# Autodesk Inventor assembly: m3X20
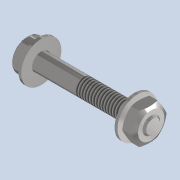
[picture p0: Inventor's stored thumbnail of the model, 180x180]
Saved by Autodesk Inventor 2020 (Build 240168000, 168)
## iProperties
Created: 2021-02-25
Part Number: m3X20
Document SubType Name: Assembly
Designer: Iulian Bors
Author: Iulian Bors
## Documents named in this file (4)
- Z:\I.A.B\Proiecte\0008 I.A.B 3D 2.1 Imprimanta aracet Metal\10 Mecanic\m3X20.iam
- Z:\I.A.B\Proiecte\0008 I.A.B 3D 2.1 Imprimanta aracet Metal\10 Mecanic\0008-10-2004 DIN 7984 - M3 x 20.ipt
- C:\Users\40743\Documents\Inventor\Content Center Files\R2020\en-US\DIN 555\DIN 555-5 - M3.ipt
- Z:\I.A.B\Proiecte\0008 I.A.B 3D 2.1 Imprimanta aracet Metal\10 Mecanic\0008-10-2005 DIN 125 - A 3.2.ipt
## Components (4 placed, 3 different names)
1. 0008-10-2004 DIN 7984 - M3 x 20.ipt:1 — Insert:1, Insert:2
2. DIN 555-5 - M3.ipt:2 — Insert:1, Insert:3
3. 0008-10-2005 DIN 125 - A 3.2.ipt:3 — Insert:2
4. 0008-10-2005 DIN 125 - A 3.2.ipt:4 — Insert:3
## Relationships (3: Insert 3)
- Insert:1: 0008-10-2004 DIN 7984 - M3 x 20.ipt:1 ↔ DIN 555-5 - M3.ipt:2
- Insert:2: 0008-10-2004 DIN 7984 - M3 x 20.ipt:1 ↔ 0008-10-2005 DIN 125 - A 3.2.ipt:3
- Insert:3: DIN 555-5 - M3.ipt:2 ↔ 0008-10-2005 DIN 125 - A 3.2.ipt:4
